# Autodesk Inventor assembly: Bearing Support
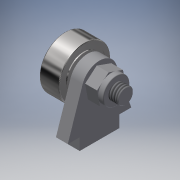
[picture p0: Inventor's stored thumbnail of the model, 180x180]
Saved by Autodesk Inventor 2018 (Build 220112000, 112)
## iProperties
Created: 2018-06-26
Part Number: Bearing Support
Document SubType Name: Assembly
Designer: Ajith Thomas
Author: Ajith Thomas
## Documents named in this file (6)
- C:\Users\Ajith Thomas\Dropbox\Gas_Sensing_Robot\FumeBot-Design\Pan and tilt assembly\Bearing Support.iam
- C:\Users\Ajith Thomas\Dropbox\Gas_Sensing_Robot\FumeBot-Design\Bearing.ipt
- C:\Users\Ajith Thomas\Dropbox\Gas_Sensing_Robot\FumeBot-Design\Pan and tilt assembly\Washers 4mm.ipt
- C:\Users\Ajith Thomas\Dropbox\Gas_Sensing_Robot\FumeBot-Design\Pan and tilt assembly\Bearing risers.ipt
- C:\Users\Ajith Thomas\Dropbox\Gas_Sensing_Robot\FumeBot-Design\Pan and tilt assembly\Bolt 4 mm x 16 mm.ipt
- C:\Users\Ajith Thomas\Dropbox\Gas_Sensing_Robot\FumeBot-Design\Pan and tilt assembly\Nut 4mm self locking.ipt
## Components (6 placed, 5 different names)
1. Bearing:1 — Flush:1, Insert:1
2. Washers 4mm:1 — Flush:1, Flush:2
3. Washers 4mm:2 — Insert:1, Insert:2
4. Bearing risers:1 — Flush:2, Insert:3
5. Bolt 4 mm x 16 mm:1 — Insert:2
6. Nut 4mm self locking:1 — Insert:3
## Relationships (5: Insert 3, Flush 2)
- Flush:1: Bearing:1 ↔ Washers 4mm:1
- Insert:1: Bearing:1 ↔ Washers 4mm:2
- Flush:2: Washers 4mm:1 ↔ Bearing risers:1
- Insert:2: Washers 4mm:2 ↔ Bolt 4 mm x 16 mm:1
- Insert:3: Bearing risers:1 ↔ Nut 4mm self locking:1
